# Autodesk Inventor assembly: TransmissionPuileyCenter
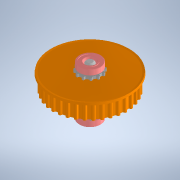
[picture p0: Inventor's stored thumbnail of the model, 180x180]
Saved by Autodesk Inventor 2022.2 (Build 262287000, 287)
## iProperties
Created: 2022-01-08
Part Number: TransmissionPuileyCenter
Document SubType Name: Assembly
Designer: Jochen
Author: Jochen
## Documents named in this file (5)
- D:\Projects\Chewbacca\CAD\Common\Motor\TransmissionPuileyCenter.iam
- D:\Projects\Chewbacca\CAD\Common\Motor\TransmissionPulleyCentreAxis.ipt
- D:\Projects\Chewbacca\CAD\Common\Motor\TransmissionCenterBigPulley.ipt
- D:\Projects\Chewbacca\CAD\Common\Motor\bearing_8_4_2_sbn_MR84VA.ipt
- D:\Projects\Chewbacca\CAD\Common\Washer\Washer m2.5.ipt
## Components (6 placed, 4 different names)
1. MotorBeltTensionerAxis:1 — Mate:1, Mate:2, Mate:3, Mate:6, Mate:7, Mate:10
2. Synchronous Pulley2:1 — Mate:1, Mate:8, Mate:11
3. bearing_8_4_2_sbn_MR84VA:1 — Mate:2, Mate:6, Mate:9
4. bearing_8_4_2_sbn_MR84VA:2 — Mate:3, Mate:12
5. Washer m2.5:1 — Mate:10, Mate:11, Mate:12
6. Washer m2.5:2 — Mate:7, Mate:8, Mate:9
## Relationships (10: Mate 10)
- Mate:1: MotorBeltTensionerAxis:1 ↔ Synchronous Pulley2:1
- Mate:2: MotorBeltTensionerAxis:1 ↔ bearing_8_4_2_sbn_MR84VA:1
- Mate:3: MotorBeltTensionerAxis:1 ↔ bearing_8_4_2_sbn_MR84VA:2
- Mate:6: MotorBeltTensionerAxis:1 ↔ bearing_8_4_2_sbn_MR84VA:1
- Mate:7: MotorBeltTensionerAxis:1 ↔ Washer m2.5:2
- Mate:8: Synchronous Pulley2:1 ↔ Washer m2.5:2
- Mate:9: bearing_8_4_2_sbn_MR84VA:1 ↔ Washer m2.5:2
- Mate:10: MotorBeltTensionerAxis:1 ↔ Washer m2.5:1
- Mate:11: Synchronous Pulley2:1 ↔ Washer m2.5:1
- Mate:12: bearing_8_4_2_sbn_MR84VA:2 ↔ Washer m2.5:1
